# Autodesk Inventor assembly: 000-base_wheel-v1
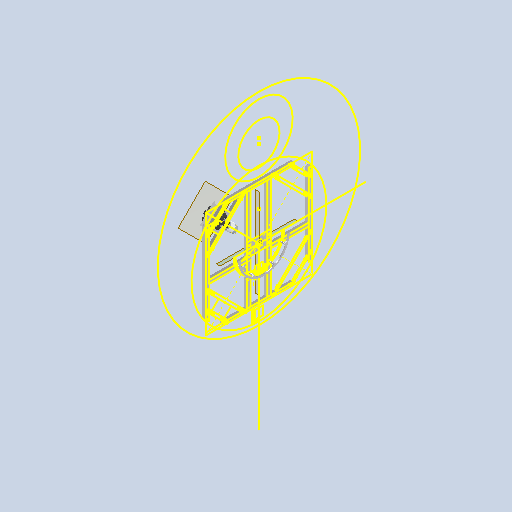
[picture p0: Inventor's stored thumbnail of the model, 512x512]
Saved by Autodesk Inventor 2025.2 (Build 292293000, 293)
## iProperties
Created: 2025-01-06
Part Number: 000-base_wheel-v1
Document SubType Name: Assembly
Designer: haruy
Author: haruy
## Documents named in this file (15)
- C:\Users\haruy\Documents\ロボコン\NHK2025\cad\nagahisa\base_weel\000-base_wheel-v1.iam
- C:\Users\haruy\Documents\ロボコン\NHK2025\cad\nagahisa\base_weel\base_weel-v2-ASP-Base.ipt
- C:\Users\haruy\Documents\ロボコン\NHK2025\cad\nagahisa\base_weel\base_weel-v2-Plate-1.ipt
- C:\Users\haruy\Documents\ロボコン\NHK2025\cad\nagahisa\base_weel\C-FL6904ZZ.ipt
- C:\Users\haruy\Documents\ロボコン\NHK2025\cad\nagahisa\base_weel\base_weel-v1-Shaft-spesa-1.ipt
- C:\Users\haruy\Documents\ロボコン\NHK2025\cad\nagahisa\base_weel\base_weel-v2-Plate-2.ipt
- C:\Users\haruy\Documents\ロボコン\NHK2025\cad\nagahisa\base_weel\takagi_weel\Workspaces\作業スペース\takagi\omuni_wheel_ver3.0\parts\omu_al_jo_1.ipt
- C:\Users\haruy\Documents\ロボコン\NHK2025\cad\nagahisa\base_weel\takagi_weel\Workspaces\作業スペース\takagi\omuni_wheel_ver3.0\parts\omu_al_jo_3.ipt
- C:\Users\haruy\Documents\ロボコン\NHK2025\cad\nagahisa\base_weel\takagi_weel\Workspaces\作業スペース\takagi\omuni_wheel_ver3.0\parts\frequently used parts\モーター\RS775\rs775_4.iam
- C:\Users\haruy\Documents\ロボコン\NHK2025\cad\nagahisa\base_weel\takagi_weel\Workspaces\作業スペース\takagi\omuni_wheel_ver3.0\parts\frequently used parts\セットカラー\SSCSP12-10\SSCSP12-10.iam
- C:\Users\haruy\Documents\ロボコン\NHK2025\cad\nagahisa\base_weel\takagi_weel\Workspaces\作業スペース\takagi\omuni_wheel_ver3.0\parts\omu_al_jo_2.ipt
- C:\Users\haruy\Documents\ロボコン\NHK2025\cad\nagahisa\base_weel\takagi_weel\Workspaces\作業スペース\takagi\omuni_wheel_ver3.0\parts\omu_sh_jo_2.ipt
- C:\Users\haruy\Documents\ロボコン\NHK2025\cad\nagahisa\base_weel\takagi_weel\Workspaces\作業スペース\takagi\omuni_wheel_ver3.0\parts\omu_sh_jo_3.ipt
- C:\Users\haruy\Documents\ロボコン\NHK2025\cad\nagahisa\base_weel\takagi_weel\Workspaces\作業スペース\takagi\omuni_wheel_ver3.0\parts\frequently used parts\ベアリング\B6201ZZNR\bearingB6201ZZNR.ipt
- C:\Users\haruy\Documents\ロボコン\NHK2025\cad\nagahisa\base_weel\takagi_weel\Workspaces\作業スペース\takagi\omuni_wheel_ver3.0\parts\frequently used parts\タイヤ\omni wheel\100mm wheel\100mm omuniwheel_MIR1.iam
## Components (21 placed, 14 different names)
1. base_weel-v2-ASP-Base:1 — 挿入:1, 挿入:2, 挿入:4, 挿入:6, 挿入:8, 挿入:9, 挿入:10, 挿入:11, 挿入:12, 挿入:13, 角度:1
2. base_weel-v2-Plate-1:1 — 挿入:1, 挿入:2, 挿入:3
3. C-FL6904ZZ:1 — 挿入:3
4. base_weel-v1-Shaft-spesa-1:1 — 挿入:4, 挿入:5
5. base_weel-v2-Plate-2:1 — 挿入:5, 挿入:7
6. base_weel-v1-Shaft-spesa-1:2 — 挿入:6, 挿入:7
7. base_weel-v1-Shaft-spesa-1:3 — 挿入:8
8. base_weel-v1-Shaft-spesa-1:4 — 挿入:9
9. omu_al_jo_1:1 — 挿入:10, 挿入:11, 挿入:20, 挿入:21, 挿入:23
10. omu_al_jo_3:1 — 挿入:12, 挿入:13, 挿入:22
11. rs775_4:1 [sub-assembly]
12. SSCSP12-10:1 [sub-assembly]
13. omu_al_jo_2:1
14. omu_sh_jo_2:1
15. omu_sh_jo_3:1 — 挿入:21
16. omu_sh_jo_3:2
17. omu_sh_jo_3:3 — 挿入:20
18. omu_sh_jo_3:4
19. bearingB6201ZZNR:1 — 挿入:23, 挿入:24
20. bearingB6201ZZNR:2 — 挿入:22
21. 100mm omuniwheel_MIR1:1 [sub-assembly] — 角度:1, 挿入:24
## Relationships (29: Insert 24, Mate 4, Angle 1)
- 挿入:1 [Insert]: base_weel-v2-ASP-Base:1 ↔ base_weel-v2-Plate-1:1
- 挿入:2 [Insert]: base_weel-v2-ASP-Base:1 ↔ base_weel-v2-Plate-1:1
- 挿入:3 [Insert]: base_weel-v2-Plate-1:1 ↔ C-FL6904ZZ:1
- 挿入:4 [Insert]: base_weel-v2-ASP-Base:1 ↔ base_weel-v1-Shaft-spesa-1:1
- 挿入:5 [Insert]: base_weel-v1-Shaft-spesa-1:1 ↔ base_weel-v2-Plate-2:1
- 挿入:6 [Insert]: base_weel-v2-ASP-Base:1 ↔ base_weel-v1-Shaft-spesa-1:2
- 挿入:7 [Insert]: base_weel-v2-Plate-2:1 ↔ base_weel-v1-Shaft-spesa-1:2
- 挿入:8 [Insert]: base_weel-v2-ASP-Base:1 ↔ base_weel-v1-Shaft-spesa-1:3
- 挿入:9 [Insert]: base_weel-v2-ASP-Base:1 ↔ base_weel-v1-Shaft-spesa-1:4
- 挿入:10 [Insert]: base_weel-v2-ASP-Base:1 ↔ omu_al_jo_1:1
- 挿入:11 [Insert]: base_weel-v2-ASP-Base:1 ↔ omu_al_jo_1:1
- 挿入:12 [Insert]: base_weel-v2-ASP-Base:1 ↔ omu_al_jo_3:1
- 挿入:13 [Insert]: base_weel-v2-ASP-Base:1 ↔ omu_al_jo_3:1
- [Mate] (5 mm): rs775_4:1 ↔ SSCSP12-10:1
- [Insert]: rs775_4:1 ↔ omu_al_jo_2:1
- [Insert]: rs775_4:1 ↔ omu_al_jo_2:1
- [Mate]: SSCSP12-10:1 ↔ omu_sh_jo_2:1
- [Mate]: rs775_4:1 ↔ omu_sh_jo_2:1
- [Mate]: rs775_4:1 ↔ omu_sh_jo_2:1
- [Insert]: omu_al_jo_2:1 ↔ omu_sh_jo_3:1
- [Insert]: omu_al_jo_2:1 ↔ omu_sh_jo_3:4
- [Insert]: omu_al_jo_2:1 ↔ omu_sh_jo_3:2
- [Insert]: omu_al_jo_2:1 ↔ omu_sh_jo_3:3
- 挿入:20 [Insert]: omu_al_jo_1:1 ↔ omu_sh_jo_3:3
- 挿入:21 [Insert]: omu_al_jo_1:1 ↔ omu_sh_jo_3:1
- 挿入:22 [Insert]: omu_al_jo_3:1 ↔ bearingB6201ZZNR:2
- 挿入:23 [Insert]: omu_al_jo_1:1 ↔ bearingB6201ZZNR:1
- 角度:1 [Angle] (0 deg): base_weel-v2-ASP-Base:1 ↔ 100mm omuniwheel_MIR1:1
- 挿入:24 [Insert] (12 mm): bearingB6201ZZNR:1 ↔ 100mm omuniwheel_MIR1:1
## Named parameters: d159_d51 = 0 mm, d160_d52 = 0 mm, d161_d53 = 0 mm, d165_d57 = 0 mm, d166_d58 = 0 mm, d167_d59 = 0 mm, d168_d60 = 0 mm, d176_d40 = 0 mm, d177_d41 = 0 mm, d178_d5 = 5 mm
